# Autodesk Inventor assembly: 足裏_1_1
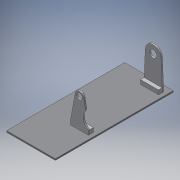
[picture p0: Inventor's stored thumbnail of the model, 180x180]
Saved by Autodesk Inventor 2018 (Build 220112000, 112)
## iProperties
Created: 2016-05-01
Part Number: 足裏_1_1
Document SubType Name: Assembly
Designer: hiroaki
Mass: 45.3916 g
Surface Area: 270.384 cm^2
Volume: 23.3732 cm^3
Density: 1.94204 g/cm^3
Author: hiroaki
## Documents named in this file (5)
- C:\Users\taka\Desktop\OPR\OpenPlatform_ver1_0\下半身\足裏\足裏_1_1_MIR.iam
- C:\Users\taka\Desktop\OPR\OpenPlatform_ver1_0\下半身\足裏\足裏_メインフレーム_1_1.ipt
- C:\Users\taka\Desktop\OPR\OpenPlatform_ver1_0\下半身\足裏\足裏_メインフレーム_1_2.ipt
- C:\Users\taka\Desktop\OPR\OpenPlatform_ver1_0\下半身\足裏\足裏_サブフレーム_1_1.ipt
- C:\Users\taka\Desktop\OPR\OpenPlatform_ver1_0\下半身\足裏\足裏_メインフレーム_1_3_MIR1.ipt
## Components (5 placed, 4 different names)
1. 足裏_メインフレーム_1_1:1 — メイト:1, フラッシュ:1, フラッシュ:2, 挿入:4, 挿入:5, 挿入:6, メイト:3
2. 足裏_メインフレーム_1_2:1 — 挿入:9, 挿入:10, メイト:3
3. 足裏_サブフレーム_1_1:1 — 挿入:9, 挿入:10, フラッシュ:3, フラッシュ:4, フラッシュ:5, フラッシュ:6, 挿入:14, 挿入:15
4. 足裏_サブフレーム_1_1:2 — 挿入:4, 挿入:5, 挿入:6, フラッシュ:3, フラッシュ:4, フラッシュ:5, フラッシュ:6, 挿入:12, 挿入:13
5. 足裏_メインフレーム_1_3_MIR1:1 — 挿入:12, 挿入:13, 挿入:14, 挿入:15
## Relationships (17: Insert 9, Flush 6, Mate 2)
- メイト:1 [Mate]: 足裏_メインフレーム_1_1:1
- フラッシュ:1 [Flush]: 足裏_メインフレーム_1_1:1
- フラッシュ:2 [Flush] (50.5 mm): 足裏_メインフレーム_1_1:1
- 挿入:4 [Insert]: 足裏_メインフレーム_1_1:1 ↔ 足裏_サブフレーム_1_1:2
- 挿入:5 [Insert]: 足裏_メインフレーム_1_1:1 ↔ 足裏_サブフレーム_1_1:2
- 挿入:6 [Insert]: 足裏_メインフレーム_1_1:1 ↔ 足裏_サブフレーム_1_1:2
- 挿入:9 [Insert]: 足裏_メインフレーム_1_2:1 ↔ 足裏_サブフレーム_1_1:1
- 挿入:10 [Insert]: 足裏_メインフレーム_1_2:1 ↔ 足裏_サブフレーム_1_1:1
- フラッシュ:3 [Flush]: 足裏_サブフレーム_1_1:1 ↔ 足裏_サブフレーム_1_1:2
- フラッシュ:4 [Flush]: 足裏_サブフレーム_1_1:1 ↔ 足裏_サブフレーム_1_1:2
- メイト:3 [Mate] (101 mm): 足裏_メインフレーム_1_1:1 ↔ 足裏_メインフレーム_1_2:1
- フラッシュ:5 [Flush]: 足裏_サブフレーム_1_1:1 ↔ 足裏_サブフレーム_1_1:2
- フラッシュ:6 [Flush]: 足裏_サブフレーム_1_1:1 ↔ 足裏_サブフレーム_1_1:2
- 挿入:12 [Insert]: 足裏_サブフレーム_1_1:2 ↔ 足裏_メインフレーム_1_3_MIR1:1
- 挿入:13 [Insert]: 足裏_サブフレーム_1_1:2 ↔ 足裏_メインフレーム_1_3_MIR1:1
- 挿入:14 [Insert]: 足裏_サブフレーム_1_1:1 ↔ 足裏_メインフレーム_1_3_MIR1:1
- 挿入:15 [Insert]: 足裏_サブフレーム_1_1:1 ↔ 足裏_メインフレーム_1_3_MIR1:1
